# Autodesk Inventor assembly: main_assembly
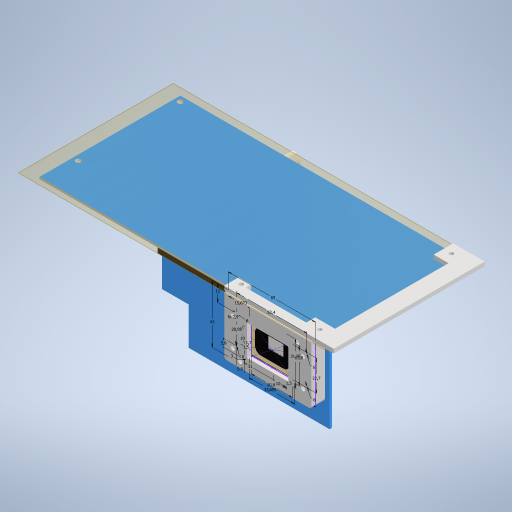
[picture p0: Inventor's stored thumbnail of the model, 512x512]
Saved by Autodesk Inventor 2024 (Build 280153000, 153)
## iProperties
Created: 2024-09-23
Part Number: main_assembly
Document SubType Name: Assembly
Designer: PC
Author: PC
## Documents named in this file (7)
- C:\Users\PC\Desktop\fotolito_czesci\main_assembly.iam
- C:\Users\PC\Desktop\fotolito_czesci\daughterboard.ipt
- C:\Users\PC\Desktop\fotolito_czesci\motherboard.ipt
- C:\Users\PC\Desktop\fotolito_czesci\tray.ipt
- C:\Users\PC\Desktop\fotolito_czesci\DLP.ipt
- C:\Users\PC\Desktop\fotolito_czesci\clamp.ipt
- C:\Users\PC\Desktop\fotolito_czesci\strut1.ipt
## Components (6 placed, 6 different names)
1. daughterboard:1 — Mate:1, Mate:2, Mate:3, Mate:5, Mate:6, Angle:1, Mate:8, Mate:9
2. motherboard:1 — Mate:1, Mate:2, Mate:3, Flush:1
3. tray:1 — Mate:5, Mate:6, Angle:1, Mate:7, Angle:2
4. DLP:1 — Mate:7, Angle:2
5. clamp:1 — Mate:8, Mate:9
6. strut1:1 — Flush:1
## Relationships (11: Mate 8, Angle 2, Flush 1)
- Mate:1: daughterboard:1 ↔ motherboard:1
- Mate:2: daughterboard:1 ↔ motherboard:1
- Mate:3 (1.75 mm): daughterboard:1 ↔ motherboard:1
- Mate:5: daughterboard:1 ↔ tray:1
- Mate:6: daughterboard:1 ↔ tray:1
- Angle:1 (0 deg): daughterboard:1 ↔ tray:1
- Mate:7: tray:1 ↔ DLP:1
- Angle:2 (0 deg): tray:1 ↔ DLP:1
- Mate:8: daughterboard:1 ↔ clamp:1
- Mate:9: daughterboard:1 ↔ clamp:1
- Flush:1: motherboard:1 ↔ strut1:1
